# Autodesk Inventor assembly: 312-01
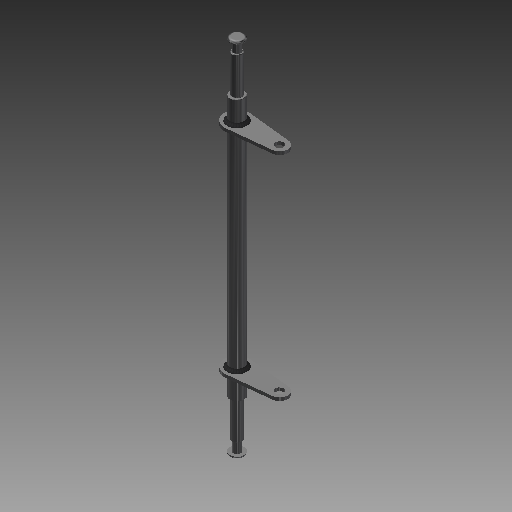
[picture p0: Inventor's stored thumbnail of the model, 512x512]
Saved by Autodesk Inventor 2019 (Build 230136000, 136)
## iProperties
Company: Autodesk Inc.
Created: 2007-10-25
Part Number: 312-01
Document SubType Name: Weldment
Designer: Autodesk Inc.
Weld Material: Welded Steel Mild (Black-Flat)
Mass: 602.959 g
Surface Area: 279.565 cm^2
Volume: 76.8087 cm^3
Density: 7.85013 g/cm^3
Description: FRONT PIVOT WELDMENT
Component Category: Lower Component
Author: Inventor
## Documents named in this file (3)
- C:\TEMP\Car Seat\Workspace\Front Pivot Weldment.iam
- C:\TEMP\Car Seat\Workspace\Pivot Bar.ipt
- C:\TEMP\Car Seat\Workspace\Front Lever.ipt
## Components (3 placed, 2 different names)
1. Pivot Bar:1 — Mate:2, Flush:2, Mate:3, Angle:1
2. Front Lever:1 — Mate:2, Flush:2, Flush:3, Angle:1
3. Front Lever:2 — Mate:3, Flush:3
## Relationships (6: Flush 3, Mate 2, Angle 1)
- Mate:2: Pivot Bar:1 ↔ Front Lever:1
- Flush:2 (25 mm): Pivot Bar:1 ↔ Front Lever:1
- Mate:3: Pivot Bar:1 ↔ Front Lever:2
- Flush:3: Front Lever:1 ↔ Front Lever:2
- [Flush] (-25 mm): Pivot Bar:1 ↔ Front Lever:2
- Angle:1 (0 deg): Pivot Bar:1 ↔ Front Lever:1
